# Autodesk Inventor assembly: lancerwheel
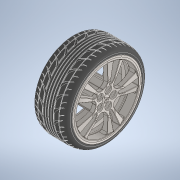
[picture p0: Inventor's stored thumbnail of the model, 180x180]
Saved by Autodesk Inventor 2021 (Build 250183000, 183)
## iProperties
Created: 2022-01-28
Part Number: lancerwheel
Document SubType Name: Assembly
Designer: juanc
Author: juanc
## Documents named in this file (3)
- C:\Users\juanc\Documents\UNAL\2021 - 2\Robótica\Proyecto\lancerwheel.iam
- C:\Users\juanc\Documents\UNAL\2021 - 2\Robótica\Proyecto\lancerrim.ipt
- C:\Users\juanc\Documents\UNAL\2021 - 2\Robótica\Proyecto\lancertire.ipt
## Components (2 placed, 2 different names)
1. lancerrim:1 — Mate:1, Mate:2
2. lancertire:1 — Mate:1, Mate:2
## Relationships (2: Mate 2)
- Mate:1: lancerrim:1 ↔ lancertire:1
- Mate:2: lancerrim:1 ↔ lancertire:1
